# Autodesk Inventor assembly: compressor tudo feito feito msmo assemblado
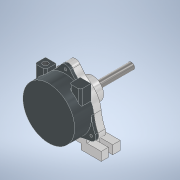
[picture p0: Inventor's stored thumbnail of the model, 180x180]
Saved by Autodesk Inventor 2022 (Build 260153000, 153)
## iProperties
Created: 2023-08-04
Part Number: compressor tudo feito feito msmo assemblado
Document SubType Name: Assembly
Designer: SENAI
Author: SENAI
## Documents named in this file (5)
- E:\TCC\compressor tudo\compressor tudo feito feito msmo assemblado.iam
- E:\TCC\compressor tudo\compressor certo certinho msmo.ipt
- E:\TCC\compressor tudo\Eixo Compressor.ipt
- E:\TCC\compressor tudo\Rotor.ipt
- E:\TCC\compressor tudo\tampa do compressor.ipt
## Components (4 placed, 4 different names)
1. compressor certo certinho msmo:1 — Mate:2, Mate:3, Mate:4
2. Eixo Compressor:1 — Mate:1, Mate:2, Flush:1
3. Rotor:1 — Mate:1, Flush:1
4. tampa do compressor:1 — Mate:3, Mate:4
## Relationships (5: Mate 4, Flush 1)
- Mate:1: Eixo Compressor:1 ↔ Rotor:1
- Mate:2: compressor certo certinho msmo:1 ↔ Eixo Compressor:1
- Flush:1: Eixo Compressor:1 ↔ Rotor:1
- Mate:3: compressor certo certinho msmo:1 ↔ tampa do compressor:1
- Mate:4: compressor certo certinho msmo:1 ↔ tampa do compressor:1
